# Autodesk Inventor assembly: dsbc-32-100-ppva-n3-3d-model-1-en_1
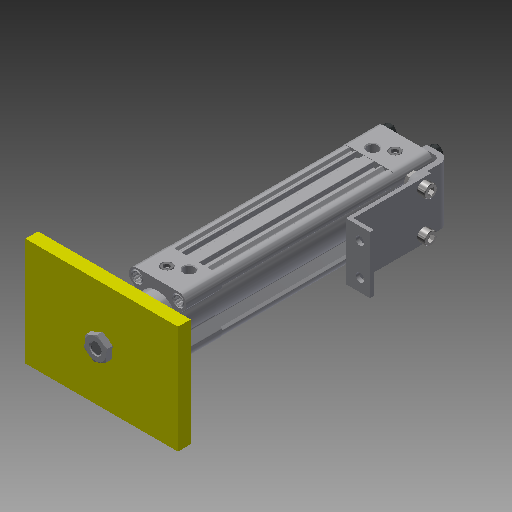
[picture p0: Inventor's stored thumbnail of the model, 512x512]
Saved by Autodesk Inventor 2019 (Build 230136000, 136)
## iProperties
Created: 2016-05-18
Part Number: dsbc-32-100-ppva-n3-3d-model-1-en_1
Description: STEP AP214
Document SubType Name: Assembly
Designer: felix
Mass: 376.574 g
Surface Area: 1269.13 cm^2
Volume: 363.299 cm^3
Density: 1.03654 g/cm^3
Sending System: PARTsolutions
Title: C:/Users/jhr/Documents/Festo/CADBasket/Export/step 2.14/d/dsbc/1376426 DSBC-32-100-PPVA-N3---(0).stp
Revision Number: NONE
## Documents named in this file (7)
- D:\Downloads\dsbc-32-100-ppva-n3-3d-model-1-en_1.iam
- D:\Downloads\HI_1463250 DSBC-32-100-PPVA_(Z).ipt
- D:\Downloads\HI_1463250 DSBC-32-100_(K).ipt
- D:\Downloads\_DIN-439-B - M10x1.25(F).ipt
- D:\Documents\Inventor\Content Center Files\Empuje2.ipt
- D:\Downloads\hnc-32-3d-model-1-en.iam
- D:\Downloads\_DIN-912 - M6x18(F).ipt
## Components (10 placed, 7 different names)
1. NAUO1 — Mate:1, Flush:1, Mate:11, Mate:12, Mate:13, Mate:14, Mate:15, Mate:16, Mate:17, Mate:20, Mate:21
2. NAUO2 — Mate:1, Flush:1, Mate:2, Mate:5, Mate:6
3. NAUO3 — Mate:2
4. _DIN-439-B - M10x1.25(F):2 — Mate:5, Mate:7
5. Empuje2:1 — Mate:6, Mate:7
6. hnc-32-3d-model-1-en:1 [sub-assembly] — Mate:15, Mate:16, Mate:17, Mate:18, Mate:19
7. _DIN-912 - M6x18(F):1 — Mate:11, Mate:20
8. _DIN-912 - M6x18(F):2 — Mate:12, Mate:18
9. _DIN-912 - M6x18(F):3 — Mate:13, Mate:19
10. _DIN-912 - M6x18(F):4 — Mate:14, Mate:21
## Relationships (17: Mate 16, Flush 1)
- Mate:1: NAUO1 ↔ NAUO2
- Flush:1 (30 mm): NAUO1 ↔ NAUO2
- Mate:2: NAUO2 ↔ NAUO3
- Mate:5: NAUO2 ↔ _DIN-439-B - M10x1.25(F):2
- Mate:6: NAUO2 ↔ Empuje2:1
- Mate:7: _DIN-439-B - M10x1.25(F):2 ↔ Empuje2:1
- Mate:11: NAUO1 ↔ _DIN-912 - M6x18(F):1
- Mate:12: NAUO1 ↔ _DIN-912 - M6x18(F):2
- Mate:13: NAUO1 ↔ _DIN-912 - M6x18(F):3
- Mate:14: NAUO1 ↔ _DIN-912 - M6x18(F):4
- Mate:15: NAUO1 ↔ hnc-32-3d-model-1-en:1
- Mate:16: NAUO1 ↔ hnc-32-3d-model-1-en:1
- Mate:17: NAUO1 ↔ hnc-32-3d-model-1-en:1
- Mate:18: hnc-32-3d-model-1-en:1 ↔ _DIN-912 - M6x18(F):2
- Mate:19: hnc-32-3d-model-1-en:1 ↔ _DIN-912 - M6x18(F):3
- Mate:20: NAUO1 ↔ _DIN-912 - M6x18(F):1
- Mate:21: NAUO1 ↔ _DIN-912 - M6x18(F):4
